# Autodesk Inventor assembly: mesoSPIM_Steinmeyer_XYZ_stages
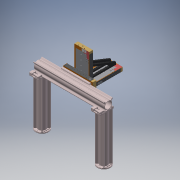
[picture p0: Inventor's stored thumbnail of the model, 180x180]
Saved by Autodesk Inventor 2016 (Build 200138000, 138)
## iProperties
Created: 2018-09-27
Part Number: mesoSPIM_Steinmeyer_XYZ_stages
Document SubType Name: Assembly
Designer: voigt
Author: voigt
## Documents named in this file (7)
- D:\Microscope_Design\CAD_Files\mesoSPIM_design\mesoSPIM\sample_stages\mesoSPIM_Steinmeyer_XYZ_stages.iam
- D:\Microscope_Design\CAD_Files\mesoSPIM_design\library\Steinmeyer_Mechatronik\PMT160-100-DCR.ipt
- D:\Microscope_Design\CAD_Files\mesoSPIM_design\library\Steinmeyer_Mechatronik\PMT160-200-DCR.ipt
- D:\Microscope_Design\CAD_Files\mesoSPIM_design\library\Thorlabs\accessoires\VB01_M_90deg_Bracket.ipt
- D:\Microscope_Design\CAD_Files\mesoSPIM_design\library\Qioptiq\X95_carriers\X95_300mm_carrier\X95_300mm_Carrier.iam
- D:\Microscope_Design\CAD_Files\mesoSPIM_design\library\Qioptiq\X95_rails\X95_750mm.ipt
- D:\Microscope_Design\CAD_Files\mesoSPIM_design\mesoSPIM\sample_stages\500mm_X95_with_base_and_clamp.iam
## Components (9 placed, 6 different names)
1. PMT160-100-DCR:1 — Mate:11, Mate:12, Mate:13, Mate:14, Mate:15, Mate:16
2. PMT160-200-DCR:1 — Mate:4, Mate:5, Angle:1, Mate:6, Mate:7, Mate:14, Mate:15, Mate:16
3. VB01_M_90deg_Bracket:1 — Mate:4, Mate:5, Angle:1, Flush:1, Mate:9
4. VB01_M_90deg_Bracket:2 — Mate:6, Mate:7, Flush:1, Mate:8, Mate:10
5. PMT160-100-DCR:2 — Mate:8, Mate:9, Mate:10
6. X95_300mm_Carrier:1 [sub-assembly] — Mate:11, Mate:12, Mate:13, Mate:17, Mate:18
7. X95_750mm:1 — Mate:17, Mate:18, Mate:19, Mate:20, Mate:21, Mate:22
8. 500mm_X95_with_base_and_clamp:1 [sub-assembly] — Mate:21, Mate:22
9. 500mm_X95_with_base_and_clamp:2 [sub-assembly] — Mate:19, Mate:20
## Relationships (21: Mate 19, Angle 1, Flush 1)
- Mate:4: PMT160-200-DCR:1 ↔ VB01_M_90deg_Bracket:1
- Mate:5: PMT160-200-DCR:1 ↔ VB01_M_90deg_Bracket:1
- Angle:1 (90 deg): PMT160-200-DCR:1 ↔ VB01_M_90deg_Bracket:1
- Mate:6: PMT160-200-DCR:1 ↔ VB01_M_90deg_Bracket:2
- Mate:7: PMT160-200-DCR:1 ↔ VB01_M_90deg_Bracket:2
- Flush:1: VB01_M_90deg_Bracket:1 ↔ VB01_M_90deg_Bracket:2
- Mate:8: VB01_M_90deg_Bracket:2 ↔ PMT160-100-DCR:2
- Mate:9: VB01_M_90deg_Bracket:1 ↔ PMT160-100-DCR:2
- Mate:10: VB01_M_90deg_Bracket:2 ↔ PMT160-100-DCR:2
- Mate:11: PMT160-100-DCR:1 ↔ X95_300mm_Carrier:1
- Mate:12: PMT160-100-DCR:1 ↔ X95_300mm_Carrier:1
- Mate:13: PMT160-100-DCR:1 ↔ X95_300mm_Carrier:1
- Mate:14: PMT160-100-DCR:1 ↔ PMT160-200-DCR:1
- Mate:15: PMT160-100-DCR:1 ↔ PMT160-200-DCR:1
- Mate:16: PMT160-100-DCR:1 ↔ PMT160-200-DCR:1
- Mate:17: X95_300mm_Carrier:1 ↔ X95_750mm:1
- Mate:18: X95_300mm_Carrier:1 ↔ X95_750mm:1
- Mate:19: X95_750mm:1 ↔ 500mm_X95_with_base_and_clamp:2
- Mate:20: X95_750mm:1 ↔ 500mm_X95_with_base_and_clamp:2
- Mate:21: X95_750mm:1 ↔ 500mm_X95_with_base_and_clamp:1
- Mate:22: X95_750mm:1 ↔ 500mm_X95_with_base_and_clamp:1
